# Autodesk Inventor assembly: Selenoid Valve 1764
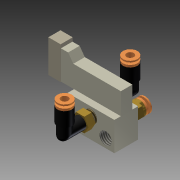
[picture p0: Inventor's stored thumbnail of the model, 180x180]
Saved by Autodesk Inventor 2011 (Build 150239000, 239)
## iProperties
Created: 2010-02-15
Part Number: Selenoid Valve 1764
Document SubType Name: Assembly
Designer: jgehrig
Author: jgehrig
## Documents named in this file (5)
- R:\CAD Archives\Pneumatics\Seloniod 1764\Selenoid Valve 1764.iam
- R:\CAD Archives\Pneumatics\Seloniod 1764\Selenoid Base 1764.ipt
- R:\CAD Archives\Pneumatics\Seloniod 1764\Selenoid Part 1764.ipt
- R:\CAD Archives\Pneumatics\Seloniod 1764\Pneumatic Screw 1764\Pneumatic Screw 1764.iam
- R:\CAD Archives\Pneumatics\Pneumatics Bend Piece 1764\Pneumatic Bend Piece 1764.iam
## Components (5 placed, 4 different names)
1. Selenoid Base 1764:1 — Flush:1, Mate:1, Flush:2, Insert:3, Insert:4, Insert:5
2. Selenoid Part 1764:1 — Flush:1, Mate:1, Flush:2, Angle:4, Angle:5
3. Pneumatic Screw 1764:1 [sub-assembly] — Insert:3
4. Pneumatic Bend Piece 1764:1 [sub-assembly] — Insert:5, Angle:4
5. Pneumatic Bend Piece 1764:2 [sub-assembly] — Insert:4, Angle:5
## Relationships (8: Insert 3, Flush 2, Angle 2, Mate 1)
- Flush:1: Selenoid Base 1764:1 ↔ Selenoid Part 1764:1
- Mate:1: Selenoid Base 1764:1 ↔ Selenoid Part 1764:1
- Flush:2 (5.715 mm): Selenoid Base 1764:1 ↔ Selenoid Part 1764:1
- Insert:3: Selenoid Base 1764:1 ↔ Pneumatic Screw 1764:1
- Insert:4: Selenoid Base 1764:1 ↔ Pneumatic Bend Piece 1764:2
- Insert:5: Selenoid Base 1764:1 ↔ Pneumatic Bend Piece 1764:1
- Angle:4 (0 deg): Selenoid Part 1764:1 ↔ Pneumatic Bend Piece 1764:1
- Angle:5 (0 deg): Selenoid Part 1764:1 ↔ Pneumatic Bend Piece 1764:2
